# Autodesk Inventor assembly: Assembly3
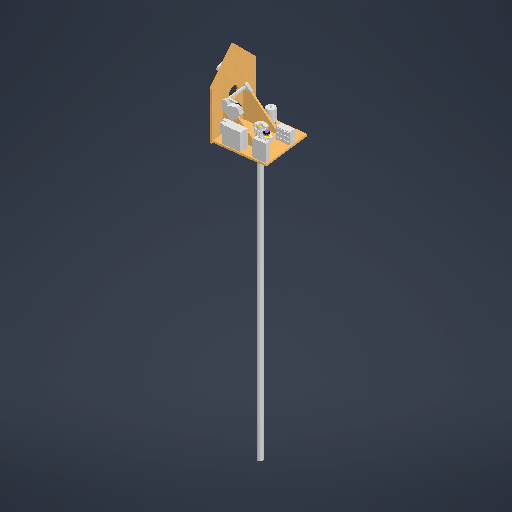
[picture p0: Inventor's stored thumbnail of the model, 512x512]
Saved by Autodesk Inventor 2026.2 (Build 302298000, 298)
## iProperties
Created: 2026-01-14
Part Number: Assembly3
Document SubType Name: Assembly
Designer: User
Author: User
## Documents named in this file (22)
- C:\Users\User\Documents\4TB6 - Capstone\Code Git\PlantMama\rev_0\Assembly3.iam
- C:\Users\User\Documents\4TB6 - Capstone\Code Git\PlantMama\rev_0\pole_v2.ipt
- C:\Users\User\Documents\4TB6 - Capstone\Code Git\PlantMama\rev_0\pole_gear_v2_with_clamp.ipt
- C:\Users\User\Documents\4TB6 - Capstone\Code Git\PlantMama\rev_0\birdhouse_holder_v1.ipt
- C:\Users\User\Documents\4TB6 - Capstone\Code Git\PlantMama\rev_0\605_2rs_bearing.ipt
- C:\Users\User\Documents\4TB6 - Capstone\Code Git\PlantMama\rev_0\pole_ring_v1_with_clamp.ipt
- C:\Users\User\Documents\4TB6 - Capstone\Code Git\PlantMama\rev_0\base_plate.ipt
- C:\Users\User\Documents\4TB6 - Capstone\Code Git\PlantMama\rev_0\drive_gear_v1.ipt
- C:\Users\User\Documents\4TB6 - Capstone\Code Git\PlantMama\rev_0\stepper_motor.ipt
- C:\Users\User\Documents\4TB6 - Capstone\Code Git\PlantMama\rev_0\side wall.ipt
- C:\Users\User\Documents\4TB6 - Capstone\Code Git\PlantMama\rev_0\front wall.ipt
- C:\Users\User\Documents\4TB6 - Capstone\Code Git\PlantMama\rev_0\turret_lift.ipt
- C:\Users\User\Documents\4TB6 - Capstone\Code Git\PlantMama\rev_0\bearing_holder_v2_left.ipt
- C:\Users\User\Documents\4TB6 - Capstone\Code Git\PlantMama\rev_0\bearing_holder_v2_right.ipt
- C:\Users\User\Documents\4TB6 - Capstone\Code Git\PlantMama\rev_0\pitch_motor_standoff_v1.ipt
- C:\Users\User\Documents\4TB6 - Capstone\Code Git\PlantMama\rev_0\pitch gear v3.ipt
- C:\Users\User\Documents\4TB6 - Capstone\Code Git\PlantMama\rev_0\temp_nozzle_v2.ipt
- C:\Users\User\Documents\4TB6 - Capstone\Code Git\PlantMama\rev_0\PowerSupply.ipt
- C:\Users\User\Documents\4TB6 - Capstone\Code Git\PlantMama\rev_0\RaspberryPi.ipt
- C:\Users\User\Documents\4TB6 - Capstone\Code Git\PlantMama\rev_0\Relay.ipt
- C:\Users\User\Documents\4TB6 - Capstone\Code Git\PlantMama\rev_0\ElectronicValve.ipt
- C:\Users\User\Documents\4TB6 - Capstone\Code Git\PlantMama\rev_0\Camera.iam
## Components (27 placed, 21 different names)
1. pole_v2:1 — Mate:2, Mate:8, Mate:9, Flush:1
2. pole_gear_v2_with_clamp:1 — Mate:9, Flush:1, Flush:2, Mate:10, Flush:3
3. birdhouse_holder_v1:1 — Mate:2, Mate:4, Mate:5, Mate:6, Mate:7, Mate:10, Mate:11, Mate:12, Mate:13
4. 605_2rs_bearing:1 — Mate:6, Mate:7
5. 605_2rs_bearing:2 — Mate:4, Mate:5, Tangent:1
6. pole_ring_v1_with_clamp:3 — Mate:8, Tangent:1, Flush:2
7. base_plate:1 — Mate:11, Mate:12, Mate:13, Flush:4, Flush:5, Mate:16, Flush:6, Flush:7, Mate:17, Flush:9, Mate:21, Mate:40, Flush:17, Mate:41, Flush:18, Flush:19, Mate:44, Flush:24, Mate:46
8. drive_gear_v1:1 — Flush:3, Mate:14, Mate:15
9. stepper_motor:1 — Mate:14, Mate:15, Flush:4, Flush:5
10. side wall:1 — Mate:16, Flush:6, Flush:7, Flush:8, Mate:18
11. front wall:1 — Mate:17, Flush:8, Flush:9, Mate:20, Mate:39, Mate:48, Mate:49, Mate:50, Mate:51
12. turret_lift:1 — Mate:18, Mate:19, Flush:10, Flush:11, Mate:20, Mate:22, Flush:12, Mate:23, Mate:26, Mate:28, Angle:2
13. turret_lift:2 — Mate:19, Flush:10, Flush:11, Mate:21, Mate:24, Flush:13, Mate:25, Mate:27, Mate:47
14. bearing_holder_v2_left:1 — Mate:22, Flush:12, Mate:23, Mate:34, Mate:35
15. bearing_holder_v2_right:1 — Mate:24, Flush:13, Mate:25
16. pitch_motor_standoff_v1:1 — Mate:26, Mate:27, Mate:28, Mate:29, Mate:30, Angle:1
17. stepper_motor:2 — Mate:29, Mate:30, Angle:1, Mate:31, Mate:32
18. drive_gear_v1:2 — Mate:31, Mate:32
19. pitch gear v3:1 — Mate:34, Mate:35, Angle:2, Mate:36, Flush:14, Mate:37
20. temp_nozzle_v2:1 — Mate:36, Flush:14, Mate:37
21. PowerSupply:1 — Mate:39, Mate:40, Flush:17
22. RaspberryPi:1 — Mate:41, Flush:18, Flush:19, Mate:45
23. Relay:1 — Flush:20, Mate:42, Flush:22, Mate:44, Flush:24, Mate:45
24. Relay:2 — Flush:20, Flush:21, Mate:42, Flush:22, Flush:23, Mate:43
25. Relay:3 — Flush:21, Flush:23, Mate:43
26. ElectronicValve:1 — Mate:46, Mate:47, Mate:48
27. Camera:1 [sub-assembly] — Mate:49, Mate:50, Mate:51
## Relationships (72: Mate 47, Flush 22, Angle 2, Tangent 1)
- Mate:2: pole_v2:1 ↔ birdhouse_holder_v1:1
- Mate:4: birdhouse_holder_v1:1 ↔ 605_2rs_bearing:2
- Mate:5: birdhouse_holder_v1:1 ↔ 605_2rs_bearing:2
- Mate:6: birdhouse_holder_v1:1 ↔ 605_2rs_bearing:1
- Mate:7: birdhouse_holder_v1:1 ↔ 605_2rs_bearing:1
- Mate:8: pole_v2:1 ↔ pole_ring_v1_with_clamp:3
- Tangent:1: 605_2rs_bearing:2 ↔ pole_ring_v1_with_clamp:3
- Mate:9: pole_v2:1 ↔ pole_gear_v2_with_clamp:1
- Flush:1: pole_v2:1 ↔ pole_gear_v2_with_clamp:1
- Flush:2: pole_gear_v2_with_clamp:1 ↔ pole_ring_v1_with_clamp:3
- Mate:10 (2 mm): pole_gear_v2_with_clamp:1 ↔ birdhouse_holder_v1:1
- Mate:11: birdhouse_holder_v1:1 ↔ base_plate:1
- Mate:12: birdhouse_holder_v1:1 ↔ base_plate:1
- Mate:13: birdhouse_holder_v1:1 ↔ base_plate:1
- Flush:3 (3 mm): pole_gear_v2_with_clamp:1 ↔ drive_gear_v1:1
- Mate:14: drive_gear_v1:1 ↔ stepper_motor:1
- Mate:15: drive_gear_v1:1 ↔ stepper_motor:1
- Flush:4 (69 mm): base_plate:1 ↔ stepper_motor:1
- Flush:5 (120 mm): base_plate:1 ↔ stepper_motor:1
- Mate:16: base_plate:1 ↔ side wall:1
- Flush:6: base_plate:1 ↔ side wall:1
- Flush:7: base_plate:1 ↔ side wall:1
- Mate:17: base_plate:1 ↔ front wall:1
- Flush:8: side wall:1 ↔ front wall:1
- Flush:9: base_plate:1 ↔ front wall:1
- Mate:18 (60 mm): side wall:1 ↔ turret_lift:1
- Mate:19 (110 mm): turret_lift:1 ↔ turret_lift:2
- Flush:10: turret_lift:1 ↔ turret_lift:2
- Flush:11: turret_lift:1 ↔ turret_lift:2
- Mate:20: front wall:1 ↔ turret_lift:1
- Mate:21: base_plate:1 ↔ turret_lift:2
- Mate:22: turret_lift:1 ↔ bearing_holder_v2_left:1
- Flush:12: turret_lift:1 ↔ bearing_holder_v2_left:1
- Mate:23: turret_lift:1 ↔ bearing_holder_v2_left:1
- Mate:24: turret_lift:2 ↔ bearing_holder_v2_right:1
- Flush:13: turret_lift:2 ↔ bearing_holder_v2_right:1
- Mate:25: turret_lift:2 ↔ bearing_holder_v2_right:1
- Mate:26: turret_lift:1 ↔ pitch_motor_standoff_v1:1
- Mate:27: turret_lift:2 ↔ pitch_motor_standoff_v1:1
- Mate:28 (150 mm): turret_lift:1 ↔ pitch_motor_standoff_v1:1
- Mate:29: pitch_motor_standoff_v1:1 ↔ stepper_motor:2
- Mate:30: pitch_motor_standoff_v1:1 ↔ stepper_motor:2
- Angle:1 (180 deg): pitch_motor_standoff_v1:1 ↔ stepper_motor:2
- Mate:31: stepper_motor:2 ↔ drive_gear_v1:2
- Mate:32: stepper_motor:2 ↔ drive_gear_v1:2
- Mate:34: bearing_holder_v2_left:1 ↔ pitch gear v3:1
- Mate:35: bearing_holder_v2_left:1 ↔ pitch gear v3:1
- Angle:2 (90 deg): turret_lift:1 ↔ pitch gear v3:1
- Mate:36: pitch gear v3:1 ↔ temp_nozzle_v2:1
- Flush:14: pitch gear v3:1 ↔ temp_nozzle_v2:1
- Mate:37 (-5 mm): pitch gear v3:1 ↔ temp_nozzle_v2:1
- Mate:39 (20 mm): front wall:1 ↔ PowerSupply:1
- Mate:40: base_plate:1 ↔ PowerSupply:1
- Flush:17 (5 mm): base_plate:1 ↔ PowerSupply:1
- Mate:41: base_plate:1 ↔ RaspberryPi:1
- Flush:18 (5 mm): base_plate:1 ↔ RaspberryPi:1
- Flush:19 (5 mm): base_plate:1 ↔ RaspberryPi:1
- Flush:20: Relay:1 ↔ Relay:2
- Flush:21: Relay:2 ↔ Relay:3
- Mate:42: Relay:1 ↔ Relay:2
- Flush:22: Relay:1 ↔ Relay:2
- Flush:23: Relay:2 ↔ Relay:3
- Mate:43: Relay:2 ↔ Relay:3
- Mate:44: base_plate:1 ↔ Relay:1
- Flush:24 (5 mm): base_plate:1 ↔ Relay:1
- Mate:45 (120 mm): RaspberryPi:1 ↔ Relay:1
- Mate:46: base_plate:1 ↔ ElectronicValve:1
- Mate:47 (20 mm): turret_lift:2 ↔ ElectronicValve:1
- Mate:48 (80 mm): front wall:1 ↔ ElectronicValve:1
- Mate:49: front wall:1 ↔ Camera:1
- Mate:50 (-280 mm): front wall:1 ↔ Camera:1
- Mate:51 (-35 mm): front wall:1 ↔ Camera:1
